# Autodesk Inventor assembly: odompod
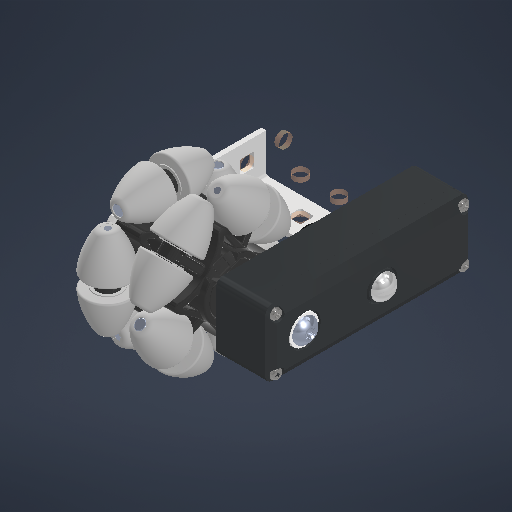
[picture p0: Inventor's stored thumbnail of the model, 512x512]
Saved by Autodesk Inventor 2026.1 (Build 301233000, 233)
## iProperties
Created: 2026-03-11
Part Number: odompod
Document SubType Name: Assembly
Designer: roejo
Author: roejo
## Documents named in this file (15)
- C:\Users\roejo\OneDrive\Documents\2026WorldChampionRobot\Robots\Worlds\Subassemblies\odompod.iam
- C:\Users\roejo\OneDrive\Documents\2026WorldChampionRobot\Library\VEX-CAD-Inventor-1.4.2\Electronics\Sensors\V5 Rotation Sensor.ipt
- C:\Users\roejo\OneDrive\Documents\2026WorldChampionRobot\Library\VEX-CAD-Inventor-1.4.2\Motion\Spacers\Washer Teflon\TWasher .375 OD x .06250.ipt
- C:\Users\roejo\OneDrive\Documents\2026WorldChampionRobot\Library\VEX-CAD-Inventor-1.4.2\Motion\Spacers\Washer Teflon.ipt
- C:\Users\roejo\OneDrive\Documents\2026WorldChampionRobot\Library\VEX-CAD-Inventor-1.4.2\Motion\Shaft HS\HS Spacer\HSpacer .1250.ipt
- C:\Users\roejo\OneDrive\Documents\2026WorldChampionRobot\Library\VEX-CAD-Inventor-1.4.2\Motion\Shaft HS\HS Spacer.ipt
- C:\Users\roejo\OneDrive\Documents\2026WorldChampionRobot\Library\VEX-CAD-Inventor-1.4.2\Motion\Wheels\Omni Wheel\2 Omni AS, No Insert.ipt
- C:\Users\roejo\OneDrive\Documents\2026WorldChampionRobot\Library\VEX-CAD-Inventor-1.4.2\Motion\Shaft HS\HS Spacer\HSpacer .0625.ipt
- C:\Users\roejo\OneDrive\Documents\2026WorldChampionRobot\Library\VEX-CAD-Inventor-1.4.2\Structure\Hardware\Screw Aluminum - Flat Head\AScrew Flat Head Threaded .500.ipt
- C:\Users\roejo\OneDrive\Documents\2026WorldChampionRobot\Library\VEX-CAD-Inventor-1.4.2\Structure\Hardware\Screw Steel - Star.ipt
- C:\Users\roejo\OneDrive\Documents\2026WorldChampionRobot\Library\VEX-CAD-Inventor-1.4.2\Structure\Hardware\Screw Steel - Star\SScrew Star Smooth 1.500.ipt
- C:\Users\roejo\OneDrive\Documents\2026WorldChampionRobot\Library\VEX-CAD-Inventor-1.4.2\Structure\Hardware\Screw Aluminum - Flat Head\AScrew Flat Head Threaded 1.000.ipt
- C:\Users\roejo\OneDrive\Documents\2026WorldChampionRobot\Library\VEX-CAD-Inventor-1.4.2\Structure\Hardware\Nut Nylon\Nut Nylon - Black.ipt
- C:\Users\roejo\OneDrive\Documents\2026WorldChampionRobot\Library\VEX-CAD-Inventor-1.4.2\Structure\Hardware\Nut Nylon.ipt
- C:\Users\roejo\OneDrive\Documents\2026WorldChampionRobot\Library\Custom Parts\odomstructure4holes.ipt
## Components (12 placed, 10 different names)
1. odomstructure4holes:1 — Insert:1, Angle:1, Insert:9, Insert:12
2. V5 Rotation Sensor:1 — Insert:1, Angle:1, Insert:2, Insert:6, Insert:11
3. TWasher .375 OD x .06250:1 — Insert:2, Insert:10
4. 2 Omni AS, No Insert:1 — Insert:4, Angle:2, Insert:8
5. 2 Omni AS, No Insert:2 — Insert:4, Angle:2, Insert:7
6. HSpacer .0625:1 — Insert:5, Insert:6
7. HSpacer .1250:2 — Insert:5, Insert:7
8. TWasher .375 OD x .06250:2 — Insert:8
9. AScrew Flat Head Threaded .500:1 — Insert:9
10. SScrew Star Smooth 1.500:1 — Insert:10
11. AScrew Flat Head Threaded 1.000:1 — Insert:11
12. Nut Nylon - Black:1 — Insert:12
## Relationships (13: Insert 11, Angle 2)
- Insert:1: odomstructure4holes:1 ↔ V5 Rotation Sensor:1
- Angle:1 (0 deg): odomstructure4holes:1 ↔ V5 Rotation Sensor:1
- Insert:2: V5 Rotation Sensor:1 ↔ TWasher .375 OD x .06250:1
- Insert:4: 2 Omni AS, No Insert:1 ↔ 2 Omni AS, No Insert:2
- Angle:2 (0 deg): 2 Omni AS, No Insert:1 ↔ 2 Omni AS, No Insert:2
- Insert:5: HSpacer .0625:1 ↔ HSpacer .1250:2
- Insert:6: V5 Rotation Sensor:1 ↔ HSpacer .0625:1
- Insert:7: 2 Omni AS, No Insert:2 ↔ HSpacer .1250:2
- Insert:8: 2 Omni AS, No Insert:1 ↔ TWasher .375 OD x .06250:2
- Insert:9: odomstructure4holes:1 ↔ AScrew Flat Head Threaded .500:1
- Insert:10: TWasher .375 OD x .06250:1 ↔ SScrew Star Smooth 1.500:1
- Insert:11: V5 Rotation Sensor:1 ↔ AScrew Flat Head Threaded 1.000:1
- Insert:12: odomstructure4holes:1 ↔ Nut Nylon - Black:1
